# Autodesk Inventor assembly: 8617.540
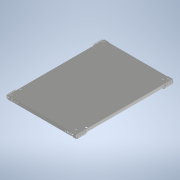
[picture p0: Inventor's stored thumbnail of the model, 180x180]
Saved by Autodesk Inventor 2021 (Build 250183000, 183)
## iProperties
Category: PARTsolutions
Company: RITTAL
Created: 2026-08-04
Part Number: 8617.540
Catalog Web Link: www.3dfindit.com
Description: VX Partial mounting plate-VX Partial mounting plate
Vendor: RITTAL
Document SubType Name: Assembly
Designer: psAdmin
Manufacturer: RITTAL
Mass: 1100.81 g
Surface Area: 8922.76 cm^2
Volume: 1100.81 cm^3
Density: 1 g/cm^3
Title: 8617.540
Author: Cadenas PARTsolutions
Comments: VX Partial mounting plate
PSOL_IDENT_0: {$CADENAS_DATA/23d-libs/rittal/sys_zub/innenausbau/montageplatten/teilmontageplatten_m51_asmtab.prj}
PSOL_IDENT_1: ,189 {VTYP=3D},{STYP=ASSTAB},{NB=8617.540},{LINA=8617.540},{NN=VX Partial mounting plate},{DATE=27.0
PSOL_IDENT_2: 7.2026 05:56:15},{GEOMDATE=27.07.2026 05:48:11},{VERSION=},{LINEID=40},{WBVAR=},{WBNUMERIC=}  {NB=86
PSOL_IDENT_3: 17.540},{LINA=8617.540},{KT=DUMMY},{BEST=8617.540},{INFOWWW=Website},{BEZ1=VX Teilmontageplatte},{BE
PSOL_IDENT_4: Z2=für neues Großschranksystem},{B=600},{BB=499},{H=800},{HH=699},{SB=600},{SH=800},{AB=600 x 800},{
PSOL_IDENT_5: VE=1},{VERS=4},{INFOPAGE=hb35_s707},{INFOPATH=http://www.rittal.com/com-en/part/8617540},{GEW=9,22},
PSOL_IDENT_6: {CNSECLASS51=27-18-92-31},{CNSECLASS70=27-40-92-16},{CNSECLASS80=27-40-92-16},{CNSETIM40=EC000213},{
PSOL_IDENT_7: BEZ3=},{DETAIL=1},{ADDGEO=1},{PPATH=assemblies/teilmontageplatten_m51_asmtpl.prj},{BESTE1=8617},{BES
PSOL_IDENT_8: TE2=540},{CNSETIM80=EC000213},{CNSETIM90=EC000213},{CNSECLASS60=27-40-92-16},{UNSPSC=31-26-15-02}
NB: 8617.540
NN: VX Partial mounting plate
NT: VX Partial mounting plate
NBSYN: $BEST.
LINA: 8617.540
CATALOG: Rittal
BEST: 8617.540
INFOWWW: webseite
BEZ1: VX Partial mounting plate
BB: 499
HH: 699
SB: 600
SH: 800
GEW: 9,22
CNSECLASS70: 27-40-92-16
CNSECLASS80: 27-40-92-16
CNSETIM80: EC000213
CNSETIM90: EC000213
CNSECLASS60: 27-40-92-16
UNSPSC: 31-26-15-02
SUPPLIER: RITTAL
ARTICLENO: 8617.540
BOMINFO: 8617.540
CREATOR: CADENAS GmbH
## Documents named in this file (5)
- e:\temp\worker_COMMON_353\temp\tmp_1132_2_wdTIU\format_0\8617_540.iam
- e:\temp\worker_COMMON_353\temp\tmp_1132_2_wdTIU\format_0\8617_540_P1.ipt
- e:\temp\worker_COMMON_353\temp\tmp_1132_2_wdTIU\format_0\8617_540_P2.ipt
- e:\temp\worker_COMMON_353\temp\tmp_1132_2_wdTIU\format_0\8617_540_P3.ipt
- e:\temp\worker_COMMON_353\temp\tmp_1132_2_wdTIU\format_0\8617_540_P4.ipt
## Components (13 placed, 4 different names)
1. 8617_540_P1:1 — P21_XY@1 <-> P21_XY@2, P21_Z@1 <-> P21_Z@2, P21_YZ@1 <-> P21_YZ@2, P22_XY@1 <-> P22_XY@3, P22_Z@1 <-> P22_Z@3, P22_YZ@1 <-> P22_YZ@3, P23_XY@1 <-> P22_XY@4, P23_Z@1 <-> P22_Z@4, P23_YZ@1 <-> P22_YZ@4, P24_XY@1 <-> P21_XY@5, P24_Z@1 <-> P21_Z@5, P24_YZ@1 <-> P21_YZ@5, P31_XY@1 <-> P3_XY@6, P31_Z@1 <-> P3_Z@6, P31_YZ@1 <-> P3_YZ@6, P32_XY@1 <-> P3_XY@8, P32_Z@1 <-> P3_Z@8, P32_YZ@1 <-> P3_YZ@8, P33_XY@1 <-> P3_XY@10, P33_Z@1 <-> P3_Z@10, P33_YZ@1 <-> P3_YZ@10, P34_XY@1 <-> P3_XY@12, P34_Z@1 <-> P3_Z@12, P34_YZ@1 <-> P3_YZ@12
2. 8617_540_P2:1 — P21_XY@1 <-> P21_XY@2, P21_Z@1 <-> P21_Z@2, P21_YZ@1 <-> P21_YZ@2
3. 8617_540_P2:2 — P22_XY@1 <-> P22_XY@3, P22_Z@1 <-> P22_Z@3, P22_YZ@1 <-> P22_YZ@3
4. 8617_540_P2:3 — P23_XY@1 <-> P22_XY@4, P23_Z@1 <-> P22_Z@4, P23_YZ@1 <-> P22_YZ@4
5. 8617_540_P2:4 — P24_XY@1 <-> P21_XY@5, P24_Z@1 <-> P21_Z@5, P24_YZ@1 <-> P21_YZ@5
6. 8617_540_P3:1 — P31_XY@1 <-> P3_XY@6, P31_Z@1 <-> P3_Z@6, P31_YZ@1 <-> P3_YZ@6, P3_XY@6 <-> P4_XY@7, P3_Z@6 <-> P4_Z@7, P3_YZ@6 <-> P4_YZ@7
7. 8617_540_P4:1 — P3_XY@6 <-> P4_XY@7, P3_Z@6 <-> P4_Z@7, P3_YZ@6 <-> P4_YZ@7
8. 8617_540_P3:2 — P32_XY@1 <-> P3_XY@8, P32_Z@1 <-> P3_Z@8, P32_YZ@1 <-> P3_YZ@8, P3_XY@8 <-> P4_XY@9, P3_Z@8 <-> P4_Z@9, P3_YZ@8 <-> P4_YZ@9
9. 8617_540_P4:2 — P3_XY@8 <-> P4_XY@9, P3_Z@8 <-> P4_Z@9, P3_YZ@8 <-> P4_YZ@9
10. 8617_540_P3:3 — P33_XY@1 <-> P3_XY@10, P33_Z@1 <-> P3_Z@10, P33_YZ@1 <-> P3_YZ@10, P3_XY@10 <-> P4_XY@11, P3_Z@10 <-> P4_Z@11, P3_YZ@10 <-> P4_YZ@11
11. 8617_540_P4:3 — P3_XY@10 <-> P4_XY@11, P3_Z@10 <-> P4_Z@11, P3_YZ@10 <-> P4_YZ@11
12. 8617_540_P3:4 — P34_XY@1 <-> P3_XY@12, P34_Z@1 <-> P3_Z@12, P34_YZ@1 <-> P3_YZ@12, P3_XY@12 <-> P4_XY@13, P3_Z@12 <-> P4_Z@13, P3_YZ@12 <-> P4_YZ@13
13. 8617_540_P4:4 — P3_XY@12 <-> P4_XY@13, P3_Z@12 <-> P4_Z@13, P3_YZ@12 <-> P4_YZ@13
## Relationships (36: Mate 24, Angle 12)
- P21_XY@1 <-> P21_XY@2 [Mate]: 8617_540_P1:1 ↔ 8617_540_P2:1
- P21_Z@1 <-> P21_Z@2 [Mate]: 8617_540_P1:1 ↔ 8617_540_P2:1
- P21_YZ@1 <-> P21_YZ@2 [Angle] (0 deg): 8617_540_P1:1 ↔ 8617_540_P2:1
- P22_XY@1 <-> P22_XY@3 [Mate]: 8617_540_P1:1 ↔ 8617_540_P2:2
- P22_Z@1 <-> P22_Z@3 [Mate]: 8617_540_P1:1 ↔ 8617_540_P2:2
- P22_YZ@1 <-> P22_YZ@3 [Angle] (180 deg): 8617_540_P1:1 ↔ 8617_540_P2:2
- P23_XY@1 <-> P22_XY@4 [Mate]: 8617_540_P1:1 ↔ 8617_540_P2:3
- P23_Z@1 <-> P22_Z@4 [Mate]: 8617_540_P1:1 ↔ 8617_540_P2:3
- P23_YZ@1 <-> P22_YZ@4 [Angle] (0 deg): 8617_540_P1:1 ↔ 8617_540_P2:3
- P24_XY@1 <-> P21_XY@5 [Mate]: 8617_540_P1:1 ↔ 8617_540_P2:4
- P24_Z@1 <-> P21_Z@5 [Mate]: 8617_540_P1:1 ↔ 8617_540_P2:4
- P24_YZ@1 <-> P21_YZ@5 [Angle] (180 deg): 8617_540_P1:1 ↔ 8617_540_P2:4
- P31_XY@1 <-> P3_XY@6 [Mate]: 8617_540_P1:1 ↔ 8617_540_P3:1
- P31_Z@1 <-> P3_Z@6 [Mate]: 8617_540_P1:1 ↔ 8617_540_P3:1
- P31_YZ@1 <-> P3_YZ@6 [Angle] (0 deg): 8617_540_P1:1 ↔ 8617_540_P3:1
- P3_XY@6 <-> P4_XY@7 [Mate]: 8617_540_P3:1 ↔ 8617_540_P4:1
- P3_Z@6 <-> P4_Z@7 [Mate]: 8617_540_P3:1 ↔ 8617_540_P4:1
- P3_YZ@6 <-> P4_YZ@7 [Angle] (0 deg): 8617_540_P3:1 ↔ 8617_540_P4:1
- P32_XY@1 <-> P3_XY@8 [Mate]: 8617_540_P1:1 ↔ 8617_540_P3:2
- P32_Z@1 <-> P3_Z@8 [Mate]: 8617_540_P1:1 ↔ 8617_540_P3:2
- P32_YZ@1 <-> P3_YZ@8 [Angle] (0 deg): 8617_540_P1:1 ↔ 8617_540_P3:2
- P3_XY@8 <-> P4_XY@9 [Mate]: 8617_540_P3:2 ↔ 8617_540_P4:2
- P3_Z@8 <-> P4_Z@9 [Mate]: 8617_540_P3:2 ↔ 8617_540_P4:2
- P3_YZ@8 <-> P4_YZ@9 [Angle] (0 deg): 8617_540_P3:2 ↔ 8617_540_P4:2
- P33_XY@1 <-> P3_XY@10 [Mate]: 8617_540_P1:1 ↔ 8617_540_P3:3
- P33_Z@1 <-> P3_Z@10 [Mate]: 8617_540_P1:1 ↔ 8617_540_P3:3
- P33_YZ@1 <-> P3_YZ@10 [Angle] (180 deg): 8617_540_P1:1 ↔ 8617_540_P3:3
- P3_XY@10 <-> P4_XY@11 [Mate]: 8617_540_P3:3 ↔ 8617_540_P4:3
- P3_Z@10 <-> P4_Z@11 [Mate]: 8617_540_P3:3 ↔ 8617_540_P4:3
- P3_YZ@10 <-> P4_YZ@11 [Angle] (0 deg): 8617_540_P3:3 ↔ 8617_540_P4:3
- P34_XY@1 <-> P3_XY@12 [Mate]: 8617_540_P1:1 ↔ 8617_540_P3:4
- P34_Z@1 <-> P3_Z@12 [Mate]: 8617_540_P1:1 ↔ 8617_540_P3:4
- P34_YZ@1 <-> P3_YZ@12 [Angle] (180 deg): 8617_540_P1:1 ↔ 8617_540_P3:4
- P3_XY@12 <-> P4_XY@13 [Mate]: 8617_540_P3:4 ↔ 8617_540_P4:4
- P3_Z@12 <-> P4_Z@13 [Mate]: 8617_540_P3:4 ↔ 8617_540_P4:4
- P3_YZ@12 <-> P4_YZ@13 [Angle] (0 deg): 8617_540_P3:4 ↔ 8617_540_P4:4
